# Autodesk Inventor assembly: Note ELP Camera
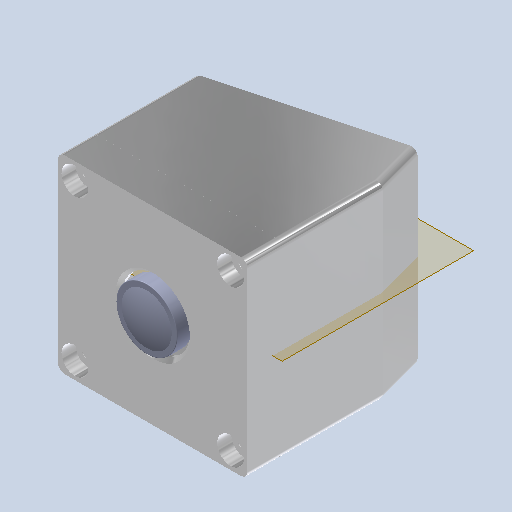
[picture p0: Inventor's stored thumbnail of the model, 512x512]
Saved by Autodesk Inventor 2023.3 (Build 273359000, 359)
## iProperties
Created: 2024-02-12
Part Number: Note ELP Camera
Document SubType Name: Assembly
Designer: mavericks
Mass: 173.621 g
Surface Area: 399.65 cm^2
Volume: 64.3041 cm^3
Density: 2.7 g/cm^3
Author: mavericks
## Documents named in this file (4)
- C:\Users\mavericks\Desktop\Crescendo_2024-CAD\2024 Robot\COMMON PARTS\ELECTRONICS\cameras\Note ELP Camera.iam
- C:\Users\mavericks\Desktop\Crescendo_2024-CAD\2024 Robot\COMMON PARTS\ELECTRONICS\cameras\ELP Camera.ipt
- C:\Users\mavericks\Desktop\Crescendo_2024-CAD\2024 Robot\COMMON PARTS\ELECTRONICS\cameras\ELP Camera Lid.ipt
- C:\Users\mavericks\Desktop\Crescendo_2024-CAD\2024 Robot\COMMON PARTS\ELECTRONICS\cameras\ELP Camera Angled' Case.ipt
## Components (3 placed, 3 different names)
1. ELP Camera Angled' Case:1
2. ELP Camera:1
3. ELP Camera Lid:1
## Relationships (6: Insert 5, Mate 1)
- [Insert]: ELP Camera Angled' Case:1 ↔ ELP Camera:1
- [Mate]: ELP Camera Angled' Case:1 ↔ ELP Camera:1
- [Insert]: ELP Camera Angled' Case:1 ↔ ELP Camera Lid:1
- [Insert]: ELP Camera Angled' Case:1 ↔ ELP Camera Lid:1
- [Insert]: ELP Camera Angled' Case:1 ↔ ELP Camera Lid:1
- [Insert]: ELP Camera Angled' Case:1 ↔ ELP Camera Lid:1
